# Autodesk Inventor assembly: 部件2
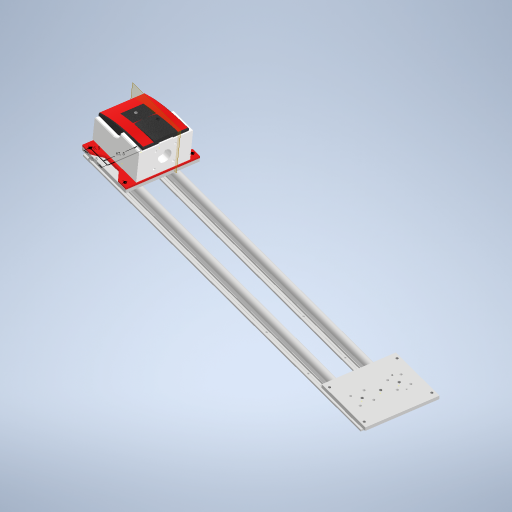
[picture p0: Inventor's stored thumbnail of the model, 512x512]
Saved by Autodesk Inventor 2023.5 (Build 275446000, 446)
## iProperties
Created: 2025-03-30
Part Number: 部件2
Document SubType Name: Assembly
Designer: jiaxue
Author: jiaxue
## Documents named in this file (6)
- C:\Users\jiaxue\Downloads\part_skcript\部件2.iam
- C:\Users\jiaxue\Downloads\part_skcript\laser_base.ipt
- C:\Users\jiaxue\Downloads\part_skcript\Adapterplatte1Gong_2025-03-28v00r00grm.ipt
- C:\Users\jiaxue\Downloads\part_skcript\Lezaj SRB20.ipt
- C:\Users\jiaxue\Downloads\part_skcript\Vodjica SBR20 L1200.ipt
- C:\Users\jiaxue\Downloads\part_skcript\Adapterplatte_messstage_Gong_2025-03-28v00r00grm.ipt
## Components (9 placed, 5 different names)
1. laser_base:1 — 配合:1, 配合:2, 配合:5, 配合:16, 配合:17
2. Adapterplatte1Gong_2025-03-28v00r00grm:1 — 配合:1, 配合:2, 配合:5, 配合:6, 配合:7, 配合:8, 配合:11, 配合:12, 配合:13, 配合:16, 配合:17
3. Lezaj SRB20:1 — 配合:6, 配合:7, 配合:8, 配合:9, 配合:10
4. Vodjica SBR20 L1200:1 — 配合:9, 配合:10, 表面齐平:1, 配合:20, 配合:21, 配合:22
5. Lezaj SRB20:2 — 配合:11, 配合:12, 配合:13, 配合:14, 配合:15
6. Vodjica SBR20 L1200:2 — 配合:14, 配合:15, 表面齐平:1, 配合:18, 配合:19
7. Lezaj SRB20:3 — 配合:18, 配合:19, 配合:23, 配合:27, 配合:28
8. Lezaj SRB20:4 — 配合:20, 配合:21, 配合:22, 配合:24
9. Adapterplatte_messstage_Gong_2025-03-28v00r00grm:1 — 配合:23, 配合:24, 配合:27, 配合:28
## Relationships (25: Mate 24, Flush 1)
- 配合:1 [Mate]: laser_base:1 ↔ Adapterplatte1Gong_2025-03-28v00r00grm:1
- 配合:2 [Mate]: laser_base:1 ↔ Adapterplatte1Gong_2025-03-28v00r00grm:1
- 配合:5 [Mate]: laser_base:1 ↔ Adapterplatte1Gong_2025-03-28v00r00grm:1
- 配合:6 [Mate]: Adapterplatte1Gong_2025-03-28v00r00grm:1 ↔ Lezaj SRB20:1
- 配合:7 [Mate]: Adapterplatte1Gong_2025-03-28v00r00grm:1 ↔ Lezaj SRB20:1
- 配合:8 [Mate]: Adapterplatte1Gong_2025-03-28v00r00grm:1 ↔ Lezaj SRB20:1
- 配合:9 [Mate] (7 mm): Lezaj SRB20:1 ↔ Vodjica SBR20 L1200:1
- 配合:10 [Mate]: Lezaj SRB20:1 ↔ Vodjica SBR20 L1200:1
- 配合:11 [Mate]: Adapterplatte1Gong_2025-03-28v00r00grm:1 ↔ Lezaj SRB20:2
- 配合:12 [Mate]: Adapterplatte1Gong_2025-03-28v00r00grm:1 ↔ Lezaj SRB20:2
- 配合:13 [Mate]: Adapterplatte1Gong_2025-03-28v00r00grm:1 ↔ Lezaj SRB20:2
- 配合:14 [Mate] (7 mm): Lezaj SRB20:2 ↔ Vodjica SBR20 L1200:2
- 配合:15 [Mate]: Lezaj SRB20:2 ↔ Vodjica SBR20 L1200:2
- 表面齐平:1 [Flush]: Vodjica SBR20 L1200:1 ↔ Vodjica SBR20 L1200:2
- 配合:16 [Mate]: laser_base:1 ↔ Adapterplatte1Gong_2025-03-28v00r00grm:1
- 配合:17 [Mate]: laser_base:1 ↔ Adapterplatte1Gong_2025-03-28v00r00grm:1
- 配合:18 [Mate] (7 mm): Vodjica SBR20 L1200:2 ↔ Lezaj SRB20:3
- 配合:19 [Mate]: Vodjica SBR20 L1200:2 ↔ Lezaj SRB20:3
- 配合:20 [Mate] (7 mm): Vodjica SBR20 L1200:1 ↔ Lezaj SRB20:4
- 配合:21 [Mate] (7 mm): Vodjica SBR20 L1200:1 ↔ Lezaj SRB20:4
- 配合:22 [Mate]: Vodjica SBR20 L1200:1 ↔ Lezaj SRB20:4
- 配合:23 [Mate]: Lezaj SRB20:3 ↔ Adapterplatte_messstage_Gong_2025-03-28v00r00grm:1
- 配合:24 [Mate]: Lezaj SRB20:4 ↔ Adapterplatte_messstage_Gong_2025-03-28v00r00grm:1
- 配合:27 [Mate]: Lezaj SRB20:3 ↔ Adapterplatte_messstage_Gong_2025-03-28v00r00grm:1
- 配合:28 [Mate]: Lezaj SRB20:3 ↔ Adapterplatte_messstage_Gong_2025-03-28v00r00grm:1
